# Autodesk Inventor assembly: SLIDE,ELEVATOR,STAGE1,LH1
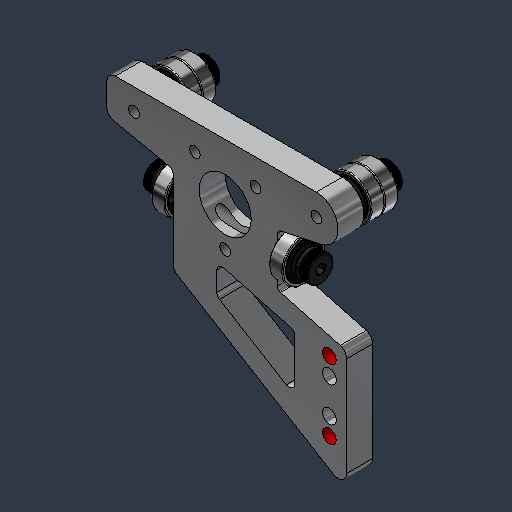
[picture p0: Inventor's stored thumbnail of the model, 512x512]
Saved by Autodesk Inventor 2024.3 (Build 283343000, 343)
## iProperties
Category: _
Manager: _
ILogicPurgeVersion: 3.4.1.0
ILogicPurgeAssembly: InventorDocumentWrapper
OnSaveVersion: 3.4.3.0
OnSaveAssembly: COREAutomationManager
Created: 2025-01-27
Part Number: SLIDE,ELEVATOR,STAGE1,LH1
Checked By: 00
Engr Approved By: _
User Status: Work In Process
Description: ASSY,STANDARD (mm)
Document SubType Name: Assembly
Mfg Approved By: John.Thibert
Designer: John.Thibert
Mass: 139.043 g
Surface Area: 267.346 cm^2
Volume: 37.8293 cm^3
Density: 3.67555 g/cm^3
CN_MASS: 0.14
CN_SERVICEABLE: _
FIRST_DESCRIPTION: _
SECOND_DESCRIPTION: _
THIRD_DESCRIPTION: _
CL_runCount: 0
ModelCat: Uncategorized
Subject: _
Author: John.Thibert
Keywords: -
Revision Number: A
## Documents named in this file (7)
- C:\Users\Jthib\OneDrive\Robotics\Poseidon\SLIDE,ELEVATOR,STAGE1,LH.iam
- C:\Users\Jthib\OneDrive\Robotics\Poseidon\PLATE,SIDE,ELEVATOR,STAGE1.ipt
- C:\Users\Jthib\OneDrive\Robotics\Poseidon\60355K336_Ball Bearing.ipt
- C:\Users\Jthib\OneDrive\Robotics\Poseidon\SPACER,BEARING,SLIDE,ELEVATOR.ipt
- C:\Users\Jthib\OneDrive\Robotics\Poseidon\91259A171_Alloy Steel Shoulder Screw.ipt
- C:\Users\Jthib\OneDrive\Robotics\Poseidon\SPACER,BEARING,SLIDE,THIN,ELEVATOR.ipt
- C:\Users\Jthib\OneDrive\Robotics\Poseidon\91259A172_Alloy Steel Shoulder Screw.ipt
## Components (15 placed, 6 different names)
1. PLATE,SIDE,ELEVATOR,STAGE1.ipt:1 — Mate:21, Mate:22, Flush:1, Insert:6, Insert:7
2. 60355K336_Ball Bearing.ipt:1
3. 60355K336_Ball Bearing.ipt:2
4. 91259A171_Alloy Steel Shoulder Screw.ipt:1
5. 91259A171_Alloy Steel Shoulder Screw.ipt:2
6. SPACER,BEARING,SLIDE,THIN,ELEVATOR.ipt:1
7. SPACER,BEARING,SLIDE,THIN,ELEVATOR.ipt:2
8. 91259A172_Alloy Steel Shoulder Screw.ipt:1 — Insert:6, Mate:23, Mate:24, Mate:26, Mate:28
9. 60355K336_Ball Bearing.ipt:3 — Mate:25, Mate:26, Mate:27
10. 60355K336_Ball Bearing.ipt:4 — Mate:23, Mate:24, Mate:25
11. SPACER,BEARING,SLIDE,ELEVATOR.ipt:1 — Mate:27, Mate:28
12. 91259A172_Alloy Steel Shoulder Screw.ipt:2 — Insert:7
13. 60355K336_Ball Bearing.ipt:5
14. 60355K336_Ball Bearing.ipt:6
15. SPACER,BEARING,SLIDE,ELEVATOR.ipt:2
## Relationships (25: Mate 18, Insert 6, Flush 1)
- [Mate]: PLATE,SIDE,ELEVATOR,STAGE1.ipt:1 ↔ 60355K336_Ball Bearing.ipt:1
- [Mate]: PLATE,SIDE,ELEVATOR,STAGE1.ipt:1 ↔ 60355K336_Ball Bearing.ipt:1
- [Mate]: PLATE,SIDE,ELEVATOR,STAGE1.ipt:1 ↔ 60355K336_Ball Bearing.ipt:2
- [Mate]: PLATE,SIDE,ELEVATOR,STAGE1.ipt:1 ↔ 60355K336_Ball Bearing.ipt:2
- [Insert]: PLATE,SIDE,ELEVATOR,STAGE1.ipt:1 ↔ 91259A171_Alloy Steel Shoulder Screw.ipt:1
- [Insert]: PLATE,SIDE,ELEVATOR,STAGE1.ipt:1 ↔ 91259A171_Alloy Steel Shoulder Screw.ipt:2
- [Insert]: 60355K336_Ball Bearing.ipt:1 ↔ SPACER,BEARING,SLIDE,THIN,ELEVATOR.ipt:1
- [Insert]: 60355K336_Ball Bearing.ipt:2 ↔ SPACER,BEARING,SLIDE,THIN,ELEVATOR.ipt:2
- Mate:21: PLATE,SIDE,ELEVATOR,STAGE1.ipt:1
- Mate:22: PLATE,SIDE,ELEVATOR,STAGE1.ipt:1
- Flush:1: PLATE,SIDE,ELEVATOR,STAGE1.ipt:1
- Insert:6: PLATE,SIDE,ELEVATOR,STAGE1.ipt:1 ↔ 91259A172_Alloy Steel Shoulder Screw.ipt:1
- Mate:23: 91259A172_Alloy Steel Shoulder Screw.ipt:1 ↔ 60355K336_Ball Bearing.ipt:4
- Mate:24: 91259A172_Alloy Steel Shoulder Screw.ipt:1 ↔ 60355K336_Ball Bearing.ipt:4
- Mate:25: 60355K336_Ball Bearing.ipt:3 ↔ 60355K336_Ball Bearing.ipt:4
- Mate:26: 91259A172_Alloy Steel Shoulder Screw.ipt:1 ↔ 60355K336_Ball Bearing.ipt:3
- Mate:27: 60355K336_Ball Bearing.ipt:3 ↔ SPACER,BEARING,SLIDE,ELEVATOR.ipt:1
- Mate:28: 91259A172_Alloy Steel Shoulder Screw.ipt:1 ↔ SPACER,BEARING,SLIDE,ELEVATOR.ipt:1
- [Mate]: 91259A172_Alloy Steel Shoulder Screw.ipt:2 ↔ 60355K336_Ball Bearing.ipt:6
- [Mate]: 91259A172_Alloy Steel Shoulder Screw.ipt:2 ↔ 60355K336_Ball Bearing.ipt:6
- [Mate]: 60355K336_Ball Bearing.ipt:5 ↔ 60355K336_Ball Bearing.ipt:6
- [Mate]: 91259A172_Alloy Steel Shoulder Screw.ipt:2 ↔ 60355K336_Ball Bearing.ipt:5
- [Mate]: 60355K336_Ball Bearing.ipt:5 ↔ SPACER,BEARING,SLIDE,ELEVATOR.ipt:2
- [Mate]: 91259A172_Alloy Steel Shoulder Screw.ipt:2 ↔ SPACER,BEARING,SLIDE,ELEVATOR.ipt:2
- Insert:7: PLATE,SIDE,ELEVATOR,STAGE1.ipt:1 ↔ 91259A172_Alloy Steel Shoulder Screw.ipt:2
## Named parameters: d92_d86 = 0 mm, d93_d87 = 0 mm, d94_d88 = 0 mm, d95_d89 = 0 mm, d96_d90 = 0 mm, d97_d91 = 0 mm
